# Autodesk Inventor assembly: righttURNwHEEL
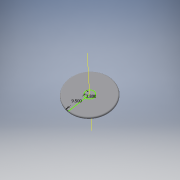
[picture p0: Inventor's stored thumbnail of the model, 180x180]
Saved by Autodesk Inventor 2018 (Build 220112000, 112)
## iProperties
Created: 2018-02-22
Part Number: righttURNwHEEL
Document SubType Name: Assembly
Designer: rochee19
Author: rochee19
## Documents named in this file (3)
- C:\Users\rochee19\Documents\righttURNwHEEL.iam
- C:\Users\rochee19\Downloads\pizza wheel.ipt
- C:\Users\rochee19\Documents\steeringBracket.ipt
## Components (2 placed, 2 different names)
1. pizza wheel:1 — Rigid:1
2. steeringBracket:1 — Rigid:1
## Relationships (1: WeldJoint 1)
- Rigid:1 [WeldJoint]: pizza wheel:1 ↔ steeringBracket:1
